# Autodesk Inventor assembly: Heating plate with 11 heating wires
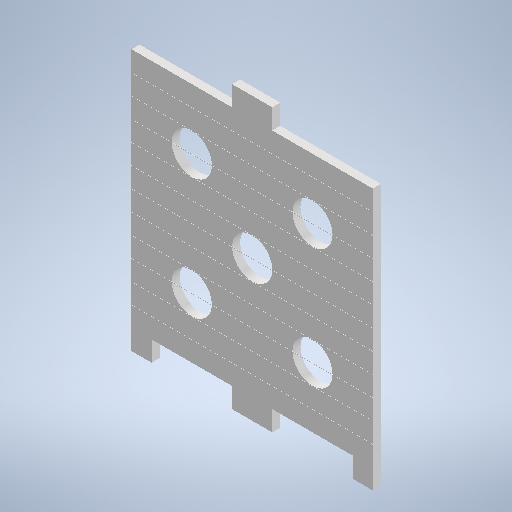
[picture p0: Inventor's stored thumbnail of the model, 512x512]
Saved by Autodesk Inventor 2025.1 (Build 291241020, 241B)
## iProperties
Created: 2024-10-29
Part Number: Heating plate with 11 heating wires
Document SubType Name: Assembly
Designer: jjk
Author: jjk
## Documents named in this file (3)
- C:\Users\jjk\Desktop\Capstone CAD\Version 2\Heating plate with 11 heating wires.iam
- C:\Users\jjk\Desktop\Capstone CAD\Version 3\Heating Plate.ipt
- C:\Users\jjk\Desktop\Capstone CAD\Version 3\flat 32 gauge nichrome wire.ipt
## Components (12 placed, 2 different names)
1. Heating Plate:1 — Flush:1, Mate:1, Flush:2
2. flat 32 gauge nichrome wire:1 — Flush:1, Mate:1, Flush:2
3. flat 32 gauge nichrome wire:2
4. flat 32 gauge nichrome wire:3
5. flat 32 gauge nichrome wire:4
6. flat 32 gauge nichrome wire:5
7. flat 32 gauge nichrome wire:6
8. flat 32 gauge nichrome wire:7
9. flat 32 gauge nichrome wire:8
10. flat 32 gauge nichrome wire:9
11. flat 32 gauge nichrome wire:10
12. flat 32 gauge nichrome wire:11
## Component patterns: (11 elements, first: flat 32 gauge nichrome wire:1)
## Relationships (3: Flush 2, Mate 1)
- Flush:1: Heating Plate:1 ↔ flat 32 gauge nichrome wire:1
- Mate:1: Heating Plate:1 ↔ flat 32 gauge nichrome wire:1
- Flush:2 (12.7 mm): Heating Plate:1 ↔ flat 32 gauge nichrome wire:1
